# Autodesk Inventor assembly: Herramienta_Final
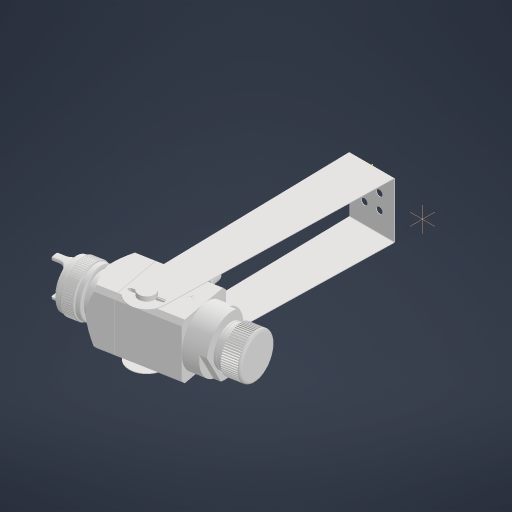
[picture p0: Inventor's stored thumbnail of the model, 512x512]
Saved by Autodesk Inventor 2024 (Build 280153000, 153)
## iProperties
Created: 2023-05-12
Part Number: Herramienta_Final
Document SubType Name: Assembly
Designer: javie
Author: javie
## Documents named in this file (3)
- C:\Users\javie\Downloads\Herramienta\Herramienta_Final.iam
- C:\Users\javie\Downloads\Herramienta\SoporteH.ipt
- C:\Users\javie\Downloads\Herramienta\Paint GunSpray.ipt
## Components (2 placed, 2 different names)
1. SoporteH:1 — Insertar:2
2. Paint GunSpray:1 — Insertar:2
## Relationships (1: Insert 1)
- Insertar:2: SoporteH:1 ↔ Paint GunSpray:1
